# Autodesk Inventor assembly: RT_MAIN_A_001
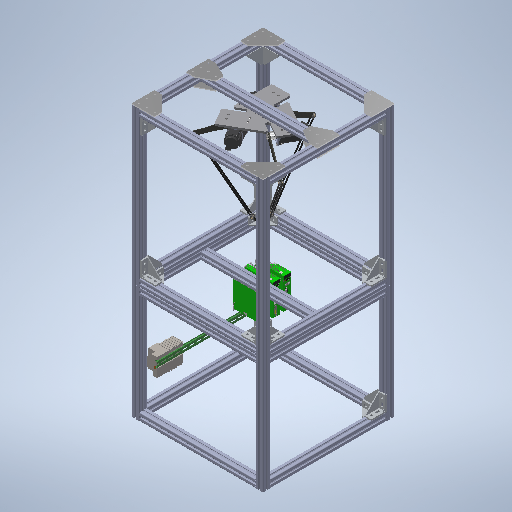
[picture p0: Inventor's stored thumbnail of the model, 512x512]
Saved by Autodesk Inventor 2025.3 (Build 293356000, 356)
## iProperties
Created: 2026-05-15
Part Number: RT_MAIN_A_001
Document SubType Name: Assembly
Designer: louis
Mass: 34530.7 g
Surface Area: 112620 cm^2
Volume: 12343.4 cm^3
Density: 2.7975 g/cm^3
Author: louis
## Documents named in this file (6)
- C:\Users\louis\OneDrive\Desktop\R_Trident\02_CAD\05_Top_Assembly\RT_MAIN_A_001.iam
- C:\Users\louis\OneDrive\Desktop\R_Trident\02_CAD\04_Subassemblies\RT_FRM_A_002_Dynamics.iam
- C:\Users\louis\OneDrive\Desktop\R_Trident\02_CAD\01_Standard_Parts\Electrical_Automation\WAGO_Din.iam
- C:\Users\louis\OneDrive\Desktop\R_Trident\02_CAD\01_Standard_Parts\A6-400EC\A6-400EC.iam
- C:\Users\louis\OneDrive\Desktop\R_Trident\02_CAD\04_Subassemblies\RT_FRM_A_003_FrameV2.iam
- C:\Users\louis\OneDrive\Desktop\R_Trident\02_CAD\04_Subassemblies\RT_FRM_A_004_ElectricalFrame.iam
## Components (7 placed, 5 different names)
1. RT_FRM_A_002_Dynamics:1 [sub-assembly] — Flush:3, Flush:4, Mate:28
2. WAGO_Din:1 [sub-assembly] — Mate:19
3. A6-400EC:1 [sub-assembly]
4. A6-400EC:2 [sub-assembly]
5. A6-400EC:3 [sub-assembly]
6. RT_FRM_A_003_FrameV2:1 [sub-assembly] — Flush:6, Flush:7, Mate:27, Flush:8, Flush:9, Flush:10, Mate:28
7. RT_FRM_A_004_ElectricalFrame:1 [sub-assembly] — Flush:6, Flush:7, Mate:27
## Relationships (12: Flush 7, Mate 5)
- Flush:3: RT_FRM_A_002_Dynamics:1
- Flush:4: RT_FRM_A_002_Dynamics:1
- Mate:16
- Mate:17
- Mate:19: WAGO_Din:1
- Flush:6: RT_FRM_A_003_FrameV2:1 ↔ RT_FRM_A_004_ElectricalFrame:1
- Flush:7: RT_FRM_A_003_FrameV2:1 ↔ RT_FRM_A_004_ElectricalFrame:1
- Mate:27: RT_FRM_A_003_FrameV2:1 ↔ RT_FRM_A_004_ElectricalFrame:1
- Flush:8: RT_FRM_A_003_FrameV2:1
- Flush:9: RT_FRM_A_003_FrameV2:1
- Flush:10: RT_FRM_A_003_FrameV2:1
- Mate:28: RT_FRM_A_002_Dynamics:1 ↔ RT_FRM_A_003_FrameV2:1
